# Autodesk Inventor assembly: Turtle Bot Assembly
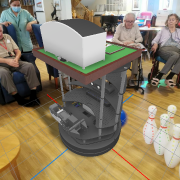
[picture p0: Inventor's stored thumbnail of the model, 180x180]
Saved by Autodesk Inventor 2021 (Build 250183000, 183)
## iProperties
Created: 2018-01-04
Part Number: Turtle Bot Assembly
Document SubType Name: Assembly
Designer: calst
Sending System: Autodesk Translation Framework v6.5.0.72
Preprocessor: ST-DEVELOPER v16.13
Title: C:/Users/setup/Desktop/Turtlebot2i.step
Author: wadecore
## Documents named in this file (18)
- C:\Users\calst\OneDrive\Desktop\University Work\Year 3\Semester 2\Integrated Group Robotics Project\Group Task\AutoDesk Inventor\TurtleBot Parts\Turtle Bot Assembly.iam
- C:\Users\calst\OneDrive\Desktop\University Work\Year 3\Semester 2\Integrated Group Robotics Project\Group Task\AutoDesk Inventor\TurtleBot Parts\standoff 50mm F_F v1.ipt
- C:\Users\calst\OneDrive\Desktop\University Work\Year 3\Semester 2\Integrated Group Robotics Project\Group Task\AutoDesk Inventor\TurtleBot Parts\BasePlate v1.ipt
- C:\Users\calst\OneDrive\Desktop\University Work\Year 3\Semester 2\Integrated Group Robotics Project\Group Task\AutoDesk Inventor\TurtleBot Parts\NUC v1.ipt
- C:\Users\calst\OneDrive\Desktop\University Work\Year 3\Semester 2\Integrated Group Robotics Project\Group Task\AutoDesk Inventor\TurtleBot Parts\MidPlateV2 v1.ipt
- C:\Users\calst\OneDrive\Desktop\University Work\Year 3\Semester 2\Integrated Group Robotics Project\Group Task\AutoDesk Inventor\TurtleBot Parts\CamPlate v1.ipt
- C:\Users\calst\OneDrive\Desktop\University Work\Year 3\Semester 2\Integrated Group Robotics Project\Group Task\AutoDesk Inventor\TurtleBot Parts\UtilPlate v1.ipt
- C:\Users\calst\OneDrive\Desktop\University Work\Year 3\Semester 2\Integrated Group Robotics Project\Group Task\AutoDesk Inventor\TurtleBot Parts\TopPlate v1.ipt
- C:\Users\calst\OneDrive\Desktop\University Work\Year 3\Semester 2\Integrated Group Robotics Project\Group Task\AutoDesk Inventor\TurtleBot Parts\Spacer M4 v1.ipt
- C:\Users\calst\OneDrive\Desktop\University Work\Year 3\Semester 2\Integrated Group Robotics Project\Group Task\AutoDesk Inventor\TurtleBot Parts\Astra v2.ipt
- C:\Users\calst\OneDrive\Desktop\University Work\Year 3\Semester 2\Integrated Group Robotics Project\Group Task\AutoDesk Inventor\TurtleBot Parts\USB Hub v4.iam
- C:\Users\calst\OneDrive\Desktop\University Work\Year 3\Semester 2\Integrated Group Robotics Project\Group Task\AutoDesk Inventor\TurtleBot Parts\Kobuki v1.ipt
- C:\Users\calst\OneDrive\Desktop\University Work\Year 3\Semester 2\Integrated Group Robotics Project\Group Task\AutoDesk Inventor\TurtleBot Parts\m3x30 standoff v1.ipt
- C:\Users\calst\OneDrive\Desktop\University Work\Year 3\Semester 2\Integrated Group Robotics Project\Group Task\AutoDesk Inventor\TurtleBot Parts\Pincher v3.iam
- C:\Users\calst\OneDrive\Desktop\University Work\Year 3\Semester 2\Integrated Group Robotics Project\Group Task\AutoDesk Inventor\TurtleBot Parts\ArbotiX-M v3.iam
- C:\Users\calst\OneDrive\Desktop\University Work\Year 3\Semester 2\Integrated Group Robotics Project\Group Task\AutoDesk Inventor\TurtleBot Parts\4500mah lipo v1.ipt
- C:\Users\calst\OneDrive\Desktop\University Work\Year 3\Semester 2\Integrated Group Robotics Project\Group Task\AutoDesk Inventor\TurtleBot Parts\OpenUPS v2.iam
- C:\Users\calst\OneDrive\Desktop\University Work\Year 3\Semester 2\Integrated Group Robotics Project\Group Task\AutoDesk Inventor\Servo\final.iam
## Components (64 placed, 17 different names)
1. standoff 50mm F/F v1:1
2. standoff 50mm F/F v1:3
3. standoff 50mm F/F v1:4
4. standoff 50mm F/F v1:6
5. standoff 50mm F/F v1:7
6. standoff 50mm F/F v1:8
7. BasePlate v1:1
8. standoff 50mm F/F v1:9
9. standoff 50mm F/F v1:10
10. standoff 50mm F/F v1:11
11. standoff 50mm F/F v1:12
12. standoff 50mm F/F v1:13
13. standoff 50mm F/F v1:14
14. NUC v1:1
15. MidPlateV2 v1:1
16. standoff 50mm F/F v1:15
17. standoff 50mm F/F v1:16
18. standoff 50mm F/F v1:17
19. standoff 50mm F/F v1:18
20. standoff 50mm F/F v1:19
21. standoff 50mm F/F v1:20
22. CamPlate v1:1
23. standoff 50mm F/F v1:27
24. standoff 50mm F/F v1:28
25. standoff 50mm F/F v1:29
26. standoff 50mm F/F v1:30
27. standoff 50mm F/F v1:31
28. standoff 50mm F/F v1:32
29. standoff 50mm F/F v1:33
30. standoff 50mm F/F v1:34
31. standoff 50mm F/F v1:35
32. standoff 50mm F/F v1:36
33. standoff 50mm F/F v1:37
34. standoff 50mm F/F v1:38
35. UtilPlate v1:1
36. standoff 50mm F/F v1:39
37. standoff 50mm F/F v1:40
38. standoff 50mm F/F v1:41
39. standoff 50mm F/F v1:42
40. standoff 50mm F/F v1:43
41. standoff 50mm F/F v1:44
42. standoff 50mm F/F v1:45
43. standoff 50mm F/F v1:46
44. standoff 50mm F/F v1:47
45. standoff 50mm F/F v1:48
46. standoff 50mm F/F v1:49
47. standoff 50mm F/F v1:50
48. TopPlate v1:1 — Mate:1
49. Spacer M4 v1:1
50. Spacer M4 v1:2
51. Spacer M4 v1:3
52. Spacer M4 v1:4
53. Astra v2:1
54. USB Hub v4:1 [sub-assembly]
55. Kobuki v1:1
56. m3x30 standoff v1:1
57. m3x30 standoff v1:2
58. m3x30 standoff v1:3
59. m3x30 standoff v1:4
60. Pincher v3:1 [sub-assembly]
61. ArbotiX-M v3:1 [sub-assembly]
62. 4500mah lipo v1:1
63. OpenUPS v2:1 [sub-assembly]
64. final:1 [sub-assembly] — Mate:1
## Relationships (1: Mate 1)
- Mate:1: TopPlate v1:1 ↔ final:1
